# Autodesk Inventor assembly: Xaxis
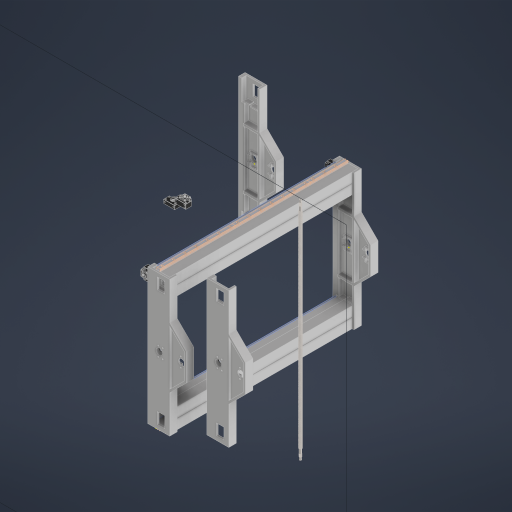
[picture p0: Inventor's stored thumbnail of the model, 512x512]
Saved by Autodesk Inventor 2024 (Build 280153000, 153)
## iProperties
Created: 2023-03-08
Part Number: Xaxis
Document SubType Name: Assembly
Designer: KirikDK
Mass: 18450.3 g
Surface Area: 38043.5 cm^2
Volume: 15460.7 cm^3
Density: 1.19337 g/cm^3
Author: KirikDK
## Documents named in this file (7)
- C:\Users\KirikDK\Documents\Stanok2023\Xaxis.iam
- C:\Users\KirikDK\Documents\Stanok2023\FlanecX_Aax.ipt
- C:\Users\KirikDK\Documents\Stanok2023\RailBlock.iam
- C:\Users\KirikDK\Documents\Stanok2023\TopZakrivka.ipt
- C:\Users\KirikDK\Documents\Stanok2023\SfuObrezki\SFU1605-600start.ipt
- C:\Users\KirikDK\Documents\Stanok2023\BF12 v1.ipt
- C:\Users\KirikDK\Documents\Stanok2023\BK12 v1.ipt
## Components (14 placed, 6 different names)
1. FlanecX_Aax:1 — Совмещение:1, Заподлицо:1, Совмещение:3, Заподлицо:2, Mate:13, Flush:6, Mate:14
2. RailBlock:2 [sub-assembly] — Совмещение:1, Заподлицо:1, Mate:8, Flush:5
3. RailBlock:3 [sub-assembly] — Совмещение:3, Заподлицо:2, Совмещение:5, Заподлицо:3, Mate:7, Flush:4
4. FlanecX_Aax:2 — Совмещение:5, Заподлицо:3, Mate:9, Mate:10, Mate:15, Flush:7, Mate:16
5. TopZakrivka:2 — Mate:8, Flush:5, Mate:10
6. TopZakrivka:3 — Mate:7, Flush:4, Mate:9
7. SFU1605-600start:1 — Mate:11, Mate:12
8. SFU1605-600start:2 — Mate:11, Mate:12
9. BF12 v1:1 — Mate:15, Flush:7, Mate:16
10. BK12 v1:1
11. BF12 v1:2
12. BK12 v1:2 — Mate:13, Flush:6, Mate:14
13. FlanecX_Aax:3
14. FlanecX_Aax:4
## Relationships (20: Mate 13, Flush 7)
- Совмещение:1 [Mate]: FlanecX_Aax:1 ↔ RailBlock:2
- Заподлицо:1 [Flush]: FlanecX_Aax:1 ↔ RailBlock:2
- Совмещение:3 [Mate]: FlanecX_Aax:1 ↔ RailBlock:3
- Заподлицо:2 [Flush]: FlanecX_Aax:1 ↔ RailBlock:3
- Совмещение:5 [Mate]: RailBlock:3 ↔ FlanecX_Aax:2
- Заподлицо:3 [Flush]: RailBlock:3 ↔ FlanecX_Aax:2
- Mate:7: RailBlock:3 ↔ TopZakrivka:3
- Mate:8: RailBlock:2 ↔ TopZakrivka:2
- Flush:4: RailBlock:3 ↔ TopZakrivka:3
- Mate:9: FlanecX_Aax:2 ↔ TopZakrivka:3
- Flush:5: RailBlock:2 ↔ TopZakrivka:2
- Mate:10: FlanecX_Aax:2 ↔ TopZakrivka:2
- Mate:11: SFU1605-600start:1 ↔ SFU1605-600start:2
- Mate:12: SFU1605-600start:1 ↔ SFU1605-600start:2
- Mate:13: FlanecX_Aax:1 ↔ BK12 v1:2
- Flush:6: FlanecX_Aax:1 ↔ BK12 v1:2
- Mate:14: FlanecX_Aax:1 ↔ BK12 v1:2
- Mate:15: FlanecX_Aax:2 ↔ BF12 v1:1
- Flush:7: FlanecX_Aax:2 ↔ BF12 v1:1
- Mate:16: FlanecX_Aax:2 ↔ BF12 v1:1
